# Autodesk Inventor assembly: Плата
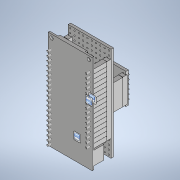
[picture p0: Inventor's stored thumbnail of the model, 180x180]
Saved by Autodesk Inventor 2020 (Build 240168000, 168)
## iProperties
Created: 2021-08-09
Part Number: Плата
Document SubType Name: Assembly
Designer: Антон
Author: Антон
## Documents named in this file (10)
- D:\Project\Robots\FutureEngineersViolet\3D-models\RRO 2021 Mk. IV\Components\Плата\Плата.iam
- D:\Project\Robots\FutureEngineersViolet\3D-models\RRO 2021 Mk. IV\Components\Плата\ESP32 LOLIN32 V1.0.0.ipt
- D:\Project\Robots\FutureEngineersViolet\3D-models\RRO 2021 Mk. IV\Components\Плата\Макетная плата 22.ipt
- D:\Project\Robots\FutureEngineersViolet\3D-models\RRO 2021 Mk. IV\Components\Плата\Гребенка 20 МАМА.ipt
- D:\Project\Robots\FutureEngineersViolet\3D-models\RRO 2021 Mk. IV\Components\Плата\Гребенка 16 МАМА.ipt
- D:\Project\Robots\FutureEngineersViolet\3D-models\RRO 2021 Mk. IV\Components\Плата\Гребенка 20 ПАПА.ipt
- D:\Project\Robots\FutureEngineersViolet\3D-models\RRO 2021 Mk. IV\Components\Плата\Гребенка 16 ПАПА.ipt
- D:\Project\Robots\FutureEngineersViolet\3D-models\RRO 2021 Mk. IV\Components\Плата\Драйвер моторов DRV8833.ipt
- D:\Project\Robots\FutureEngineersViolet\3D-models\RRO 2021 Mk. IV\Components\Плата\Гребенка 6 МАМА.ipt
- D:\Project\Robots\FutureEngineersViolet\3D-models\RRO 2021 Mk. IV\Components\Плата\Гребенка 6 ПАПА.ipt
## Components (11 placed, 5 different names)
1. ESP32 LOLIN32 V1.0.0:1 — Жесткий:1, С поворотом:1
2. Макетная плата 22*10:1 — Жесткий:2, Жесткий:5, Жесткий:10
3. Гребенка 20 МАМА:1 — Жесткий:1, Жесткий:3
4. Гребенка 20 МАМА:2 — С поворотом:1, Жесткий:4
5. Гребенка 20 ПАПА:1 — Жесткий:2, Жесткий:3
6. Гребенка 20 ПАПА:2 — Жесткий:4, Жесткий:5
7. Драйвер моторов DRV8833:1 — Жесткий:6, Жесткий:7
8. Гребенка 20 МАМА:3 — Жесткий:9
9. Гребенка 20 ПАПА:3 — Жесткий:7, Жесткий:9
10. Гребенка 20 МАМА:4 — Жесткий:8, Жесткий:10
11. Гребенка 20 ПАПА:4 — Жесткий:6, Жесткий:8
## Relationships (11: WeldJoint 10, RevoluteJoint 1)
- Жесткий:1 [WeldJoint]: ESP32 LOLIN32 V1.0.0:1 ↔ Гребенка 20 МАМА:1
- С поворотом:1 [RevoluteJoint]: ESP32 LOLIN32 V1.0.0:1 ↔ Гребенка 20 МАМА:2
- Жесткий:2 [WeldJoint] (0.4 mm): Макетная плата 22*10:1 ↔ Гребенка 20 ПАПА:1
- Жесткий:3 [WeldJoint]: Гребенка 20 МАМА:1 ↔ Гребенка 20 ПАПА:1
- Жесткий:4 [WeldJoint]: Гребенка 20 МАМА:2 ↔ Гребенка 20 ПАПА:2
- Жесткий:5 [WeldJoint] (0.4 mm): Макетная плата 22*10:1 ↔ Гребенка 20 ПАПА:2
- Жесткий:6 [WeldJoint] (-0.4 mm): Драйвер моторов DRV8833:1 ↔ Гребенка 20 ПАПА:4
- Жесткий:7 [WeldJoint] (-0.4 mm): Драйвер моторов DRV8833:1 ↔ Гребенка 20 ПАПА:3
- Жесткий:8 [WeldJoint]: Гребенка 20 МАМА:4 ↔ Гребенка 20 ПАПА:4
- Жесткий:9 [WeldJoint]: Гребенка 20 МАМА:3 ↔ Гребенка 20 ПАПА:3
- Жесткий:10 [WeldJoint]: Макетная плата 22*10:1 ↔ Гребенка 20 МАМА:4
